# Autodesk Inventor assembly: IN-12 Nixie Tube
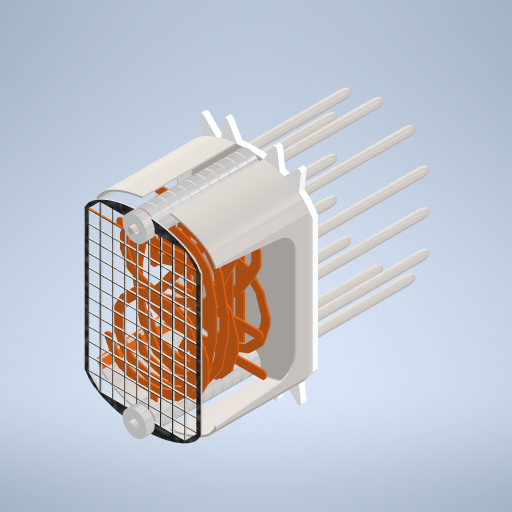
[picture p0: Inventor's stored thumbnail of the model, 512x512]
Saved by Autodesk Inventor 2024.3 (Build 283343000, 343)
## iProperties
Created: 2022-09-23
Part Number: IN-12 Nixie Tube
Description: STEP AP214
Document SubType Name: Assembly
Designer: megha
Sending System: SolidWorks 2020
Preprocessor: SwSTEP 2.0
Title: IN-12 Nixie Tube.STEP
Revision Number: ANY
## Documents named in this file (17)
- C:\Users\megha\KiCad\8.99\projects\delorean\KiCAD\libs\steps\IN-12 Nixie Tube\IN-12 Nixie Tube\IN-12 Nixie Tube.iam
- C:\Users\megha\KiCad\8.99\projects\delorean\KiCAD\libs\steps\IN-12 Nixie Tube\IN-12 Nixie Tube\IN-12 nixie tube pin.ipt
- C:\Users\megha\KiCad\8.99\projects\delorean\KiCAD\libs\steps\IN-12 Nixie Tube\IN-12 Nixie Tube\IN-12 nixie tube anode grid.ipt
- C:\Users\megha\KiCad\8.99\projects\delorean\KiCAD\libs\steps\IN-12 Nixie Tube\IN-12 Nixie Tube\IN-12 nixie tube 0 digit.ipt
- C:\Users\megha\KiCad\8.99\projects\delorean\KiCAD\libs\steps\IN-12 Nixie Tube\IN-12 Nixie Tube\IN-12 nixie tube 1 digit.ipt
- C:\Users\megha\KiCad\8.99\projects\delorean\KiCAD\libs\steps\IN-12 Nixie Tube\IN-12 Nixie Tube\IN-12 nixie tube 2 digit.ipt
- C:\Users\megha\KiCad\8.99\projects\delorean\KiCAD\libs\steps\IN-12 Nixie Tube\IN-12 Nixie Tube\IN-12 nixie tube 3 digit.ipt
- C:\Users\megha\KiCad\8.99\projects\delorean\KiCAD\libs\steps\IN-12 Nixie Tube\IN-12 Nixie Tube\IN-12 nixie tube 4 digit.ipt
- C:\Users\megha\KiCad\8.99\projects\delorean\KiCAD\libs\steps\IN-12 Nixie Tube\IN-12 Nixie Tube\IN-12 nixie tube 5 digit.ipt
- C:\Users\megha\KiCad\8.99\projects\delorean\KiCAD\libs\steps\IN-12 Nixie Tube\IN-12 Nixie Tube\IN-12 nixie tube 6 digit.ipt
- C:\Users\megha\KiCad\8.99\projects\delorean\KiCAD\libs\steps\IN-12 Nixie Tube\IN-12 Nixie Tube\IN-12 nixie tube 7 digit.ipt
- C:\Users\megha\KiCad\8.99\projects\delorean\KiCAD\libs\steps\IN-12 Nixie Tube\IN-12 Nixie Tube\IN-12 nixie tube 8 digit.ipt
- C:\Users\megha\KiCad\8.99\projects\delorean\KiCAD\libs\steps\IN-12 Nixie Tube\IN-12 Nixie Tube\IN-12 nixie tube 9 digit.ipt
- C:\Users\megha\KiCad\8.99\projects\delorean\KiCAD\libs\steps\IN-12 Nixie Tube\IN-12 Nixie Tube\IN-12 nixie tube spacer.ipt
- C:\Users\megha\KiCad\8.99\projects\delorean\KiCAD\libs\steps\IN-12 Nixie Tube\IN-12 Nixie Tube\IN-12 nixie tube rod.ipt
- C:\Users\megha\KiCad\8.99\projects\delorean\KiCAD\libs\steps\IN-12 Nixie Tube\IN-12 Nixie Tube\IN-12 nixie tube back plate 1.ipt
- C:\Users\megha\KiCad\8.99\projects\delorean\KiCAD\libs\steps\IN-12 Nixie Tube\IN-12 Nixie Tube\IN-12 nixie tube back plate 2.ipt
## Components (51 placed, 51 different names)
1. IN-12 nixie tube pin_2
2. IN-12 nixie tube pin_3
3. IN-12 nixie tube pin_4
4. IN-12 nixie tube pin_5
5. IN-12 nixie tube pin_6
6. IN-12 nixie tube pin_7
7. IN-12 nixie tube pin_8
8. IN-12 nixie tube pin_9
9. IN-12 nixie tube pin_10
10. IN-12 nixie tube pin_11
11. IN-12 nixie tube pin_12
12. IN-12 nixie tube pin_13
13. IN-12 nixie tube anode grid_14
14. IN-12 nixie tube 0 digit_15
15. IN-12 nixie tube 1 digit_16
16. IN-12 nixie tube 2 digit_17
17. IN-12 nixie tube 3 digit_18
18. IN-12 nixie tube 4 digit_19
19. IN-12 nixie tube 5 digit_20
20. IN-12 nixie tube 6 digit_21
21. IN-12 nixie tube 7 digit_22
22. IN-12 nixie tube 8 digit_23
23. IN-12 nixie tube 9 digit_24
24. IN-12 nixie tube spacer_25
25. IN-12 nixie tube spacer_26
26. IN-12 nixie tube spacer_27
27. IN-12 nixie tube spacer_28
28. IN-12 nixie tube spacer_29
29. IN-12 nixie tube spacer_30
30. IN-12 nixie tube spacer_31
31. IN-12 nixie tube spacer_32
32. IN-12 nixie tube spacer_33
33. IN-12 nixie tube spacer_34
34. IN-12 nixie tube spacer_35
35. IN-12 nixie tube spacer_36
36. IN-12 nixie tube spacer_37
37. IN-12 nixie tube spacer_38
38. IN-12 nixie tube spacer_39
39. IN-12 nixie tube spacer_40
40. IN-12 nixie tube spacer_41
41. IN-12 nixie tube spacer_42
42. IN-12 nixie tube spacer_43
43. IN-12 nixie tube spacer_44
44. IN-12 nixie tube spacer_45
45. IN-12 nixie tube spacer_46
46. IN-12 nixie tube spacer_47
47. IN-12 nixie tube spacer_48
48. IN-12 nixie tube rod_49
49. IN-12 nixie tube rod_50
50. IN-12 nixie tube back plate 1_51
51. IN-12 nixie tube back plate 2_52
## Named parameters: Finish1_Area = 5.05868, Finish2_Area = 0.720055, Finish3_Area = 0.720055, Finish4_Area = 0.438723, Finish5_Area = 3.18731, Finish6_Area = 2.38761, Finish7_Area = 0.879805
note: some values were not read from the file. Shown as the stored number, unit unknown: "Finish1_Area", "Finish2_Area", "Finish3_Area", "Finish4_Area", "Finish5_Area", "Finish6_Area", "Finish7_Area".
